# Autodesk Inventor assembly: Dog Collar Box V1.0
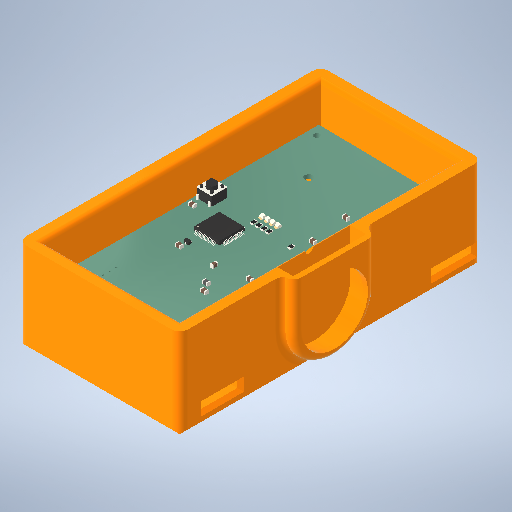
[picture p0: Inventor's stored thumbnail of the model, 512x512]
Saved by Autodesk Inventor 2025 (Build 290162000, 162)
## iProperties
Created: 2024-09-18
Part Number: Dog Collar Box V1.0
Document SubType Name: Assembly
Designer: NDurn
Author: NDurn
## Documents named in this file (5)
- C:\Users\Nick\Desktop\Github\Senior-Design-Dog-Collar\3d model\Dog Collar Box V1.0.iam
- C:\Users\Nick\Desktop\Github\Senior-Design-Dog-Collar\3d model\Battery box.ipt
- C:\Users\Nick\Desktop\Github\Senior-Design-Dog-Collar\3d model\PCB Holder.ipt
- C:\Users\Nick\Desktop\Github\Senior-Design-Dog-Collar\3d model\Lid.ipt
- C:\Users\Nick\Desktop\Github\Senior-Design-Dog-Collar\3d model\PCB\PCB.iam
## Components (4 placed, 4 different names)
1. Battery box:1 — Flush:1
2. PCB Holder:1 — Flush:1, Flush:2
3. Lid:1 — Flush:2
4. PCB:1 [sub-assembly]
## Relationships (2: Flush 2)
- Flush:1: Battery box:1 ↔ PCB Holder:1
- Flush:2: PCB Holder:1 ↔ Lid:1
